# Autodesk Inventor assembly: FemaleHeaderPin_1x4
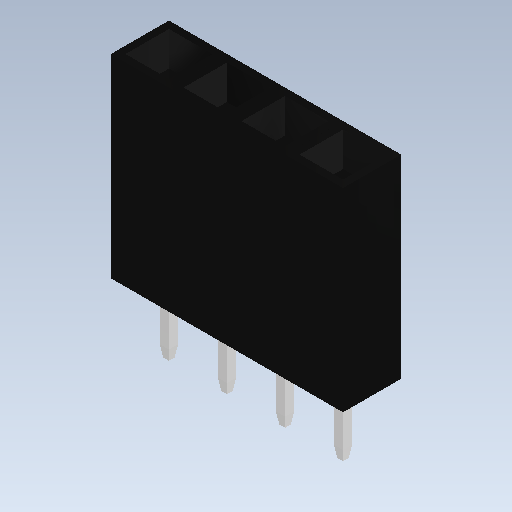
[picture p0: Inventor's stored thumbnail of the model, 512x512]
Saved by Autodesk Inventor 2020 (Build 240168000, 168)
## iProperties
Created: 2020-01-02
Part Number: FemaleHeaderPin_1x4
Document SubType Name: Assembly
Designer: ermoz
Mass: 0.213921 g
Surface Area: 4.48219 cm^2
Volume: 0.213921 cm^3
Density: 1 g/cm^3
Author: ermoz
## Documents named in this file (2)
- D:\Moje Wyczyny\Liceum\VLOat INTvators\Moje projekty\Processor Project (kontynuacja)\Drugie podejście\Electric Elements\FemaleHeaderPin_1x4.iam
- D:\Moje Wyczyny\Liceum\VLOat INTvators\Moje projekty\Processor Project (kontynuacja)\Drugie podejście\Electric Elements\FemaleHederPin.ipt
## Components (4 placed, 1 different names)
1. FemaleHederPin:1 — Mate:1, Flush:1, Flush:7
2. FemaleHederPin:2 — Mate:1, Mate:2, Flush:1, Flush:2, Flush:7, Flush:8
3. FemaleHederPin:3 — Mate:2, Mate:3, Flush:2, Flush:3, Flush:8, Flush:9
4. FemaleHederPin:4 — Mate:3, Flush:3, Flush:9
## Relationships (9: Flush 6, Mate 3)
- Mate:1: FemaleHederPin:1 ↔ FemaleHederPin:2
- Mate:2: FemaleHederPin:2 ↔ FemaleHederPin:3
- Mate:3: FemaleHederPin:3 ↔ FemaleHederPin:4
- Flush:1: FemaleHederPin:1 ↔ FemaleHederPin:2
- Flush:2: FemaleHederPin:2 ↔ FemaleHederPin:3
- Flush:3: FemaleHederPin:3 ↔ FemaleHederPin:4
- Flush:7: FemaleHederPin:1 ↔ FemaleHederPin:2
- Flush:8: FemaleHederPin:2 ↔ FemaleHederPin:3
- Flush:9: FemaleHederPin:3 ↔ FemaleHederPin:4
